# Autodesk Inventor assembly: 8042548
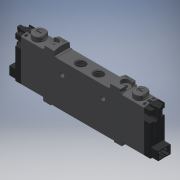
[picture p0: Inventor's stored thumbnail of the model, 180x180]
Saved by Autodesk Inventor 2017.1 (Build 211199000, 199)
## iProperties
Category: Bag #9
Company: Autodesk Inc.
Created: 2016-12-23
Part Number: 8042548
Catalog Web Link: www.festo.us/first
Description: VUVG-Solenoid valve
Vendor: FESTO
Document SubType Name: Assembly
Designer: Autodesk Inc.
Manufacturer: FESTO
Title: 8042548 VUVG-LK10-B52-T-M7-1H2L-S
Author: Autodesk Inc.
Comments: Solenoid valve
Keywords: Yellow Tote
## Documents named in this file (3)
- D:\FIRST\FIRST KOP 2017\FIRST 2017 Yellow Tote\8042548.iam
- D:\FIRST\FIRST KOP 2017\FIRST 2017 Yellow Tote\Parts\564212 VUVG-LK10-B52---T-M7--1H2--L-----(G).ipt
- D:\FIRST\FIRST KOP 2017\FIRST 2017 Yellow Tote\Parts\3779382 VUVG-LK-IP40.ipt
## Components (3 placed, 2 different names)
1. 564212 VUVG-LK10-B52---T-M7--1H2--L-----(G):1 — VAVE2_XY@1 <-> VAVE_XY@2, VAVE2_Z@1 <-> VAVE_Z@2, VAVE2_YZ@1 <-> VAVE_YZ@2, VAVE1_XY@1 <-> VAVE_XY@3, VAVE1_Z@1 <-> VAVE_Z@3, VAVE1_YZ@1 <-> VAVE_YZ@3
2. 3779382 VUVG-LK-IP40:1 — VAVE2_XY@1 <-> VAVE_XY@2, VAVE2_Z@1 <-> VAVE_Z@2, VAVE2_YZ@1 <-> VAVE_YZ@2
3. 3779382 VUVG-LK-IP40:2 — VAVE1_XY@1 <-> VAVE_XY@3, VAVE1_Z@1 <-> VAVE_Z@3, VAVE1_YZ@1 <-> VAVE_YZ@3
## Relationships (6: Mate 4, Angle 2)
- VAVE2_XY@1 <-> VAVE_XY@2 [Mate]: 564212 VUVG-LK10-B52---T-M7--1H2--L-----(G):1 ↔ 3779382 VUVG-LK-IP40:1
- VAVE2_Z@1 <-> VAVE_Z@2 [Mate]: 564212 VUVG-LK10-B52---T-M7--1H2--L-----(G):1 ↔ 3779382 VUVG-LK-IP40:1
- VAVE2_YZ@1 <-> VAVE_YZ@2 [Angle] (0 deg): 564212 VUVG-LK10-B52---T-M7--1H2--L-----(G):1 ↔ 3779382 VUVG-LK-IP40:1
- VAVE1_XY@1 <-> VAVE_XY@3 [Mate]: 564212 VUVG-LK10-B52---T-M7--1H2--L-----(G):1 ↔ 3779382 VUVG-LK-IP40:2
- VAVE1_Z@1 <-> VAVE_Z@3 [Mate]: 564212 VUVG-LK10-B52---T-M7--1H2--L-----(G):1 ↔ 3779382 VUVG-LK-IP40:2
- VAVE1_YZ@1 <-> VAVE_YZ@3 [Angle] (180 deg): 564212 VUVG-LK10-B52---T-M7--1H2--L-----(G):1 ↔ 3779382 VUVG-LK-IP40:2
